# Autodesk Inventor assembly: eh2p-00 - K3D EH2P
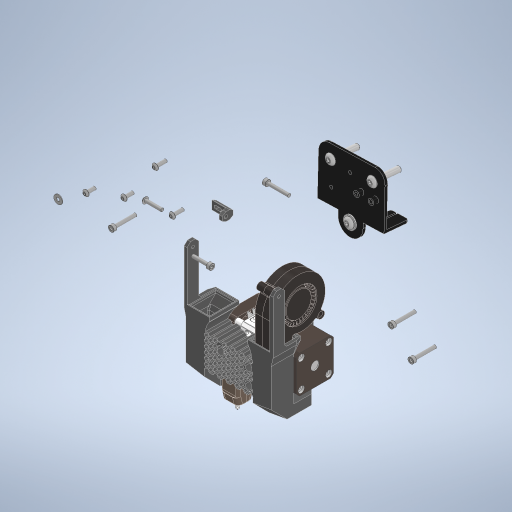
[picture p0: Inventor's stored thumbnail of the model, 512x512]
Saved by Autodesk Inventor 2024 (Build 280153000, 153)
## iProperties
Created: 2023-11-25
Part Number: eh2p-00 - K3D EH2P
Description: CAx-IF Rec.Pracs.---Representation and Presentation of Product Manufacturing Information (PMI)---4.0---2014-10-13
Document SubType Name: Assembly
Designer: wtsh
Sending System: SIEMENS PLM Software NX2306.1700
Preprocessor: ST-DEVELOPER v19.4
Title: eh2p-00 - K3D EH2P
## Documents named in this file (20)
- C:\Users\wtsh\Documents\Inventor\K3D-EHP\k3d_ehp_v2_assembly\k3d_ehp_v2_assembly.iam
- C:\Users\wtsh\Documents\Inventor\K3D-EHP\k3d_ehp_v2_assembly\Screw round M3x6.ipt
- C:\Users\wtsh\Documents\Inventor\K3D-EHP\k3d_ehp_v2_assembly\Screw socket M3x20.ipt
- C:\Users\wtsh\Documents\Inventor\K3D-EHP\k3d_ehp_v2_assembly\Screw round M5x25.ipt
- C:\Users\wtsh\Documents\Inventor\K3D-EHP\k3d_ehp_v2_assembly\eh2p-06b - United fan ducts for v6 with CRTouch.ipt
- C:\Users\wtsh\Documents\Inventor\K3D-EHP\k3d_ehp_v2_assembly\eh2p-06a - United fan ducts for v6.ipt
- C:\Users\wtsh\Documents\Inventor\K3D-EHP\k3d_ehp_v2_assembly\eh2p-05a - United fan ducts for volcano.ipt
- C:\Users\wtsh\Documents\Inventor\K3D-EHP\k3d_ehp_v2_assembly\eh2p-05b - United fan ducts for volcano with CRTouch.ipt
- C:\Users\wtsh\Documents\Inventor\K3D-EHP\k3d_ehp_v2_assembly\CR-Touch.ipt
- C:\Users\wtsh\Documents\Inventor\K3D-EHP\k3d_ehp_v2_assembly\Fan 5015.ipt
- C:\Users\wtsh\Documents\Inventor\K3D-EHP\k3d_ehp_v2_assembly\Screw round M3x16.ipt
- C:\Users\wtsh\Documents\Inventor\K3D-EHP\k3d_ehp_v2_assembly\Screw round M3x8.ipt
- C:\Users\wtsh\Documents\Inventor\K3D-EHP\k3d_ehp_v2_assembly\Nut M3.ipt
- C:\Users\wtsh\Documents\Inventor\K3D-EHP\k3d_ehp_v2_assembly\Washer M3.ipt
- C:\Users\wtsh\Documents\Inventor\K3D-EHP\k3d_ehp_v2_assembly\eh2p-02 - mount slider.ipt
- C:\Users\wtsh\Documents\Inventor\K3D-EHP\k3d_ehp_v2_assembly\h2 v2s lite.ipt
- C:\Users\wtsh\Documents\Inventor\K3D-EHP\k3d_ehp_v2_assembly\Washer M5.ipt
- C:\Users\wtsh\Documents\Inventor\K3D-EHP\k3d_ehp_v2_assembly\Screw round M3x10.ipt
- C:\Users\wtsh\Documents\Inventor\K3D-EHP\k3d_ehp_v2_assembly\eh2p-01 - H2 V2S mount (ender).ipt
- C:\Users\wtsh\Documents\Inventor\K3D-EHP\k3d_ehp_v2_assembly\Ender-3 carriage.ipt
## Components (30 placed, 19 different names)
1. Screw round M3x6 — С поворотом:1
2. Screw round M3x6:1 — С поворотом:6
3. Screw socket M3x20
4. Screw socket M3x20:1
5. Screw round M5x25 — С поворотом:5
6. Screw round M5x25:1 — С поворотом:2
7. eh2p-06b - United fan ducts for v6 with CRTouch — Жесткий:1, Совмещение:1, Угол:3, Совмещение:2, С поворотом:8
8. eh2p-06a - United fan ducts for v6
9. eh2p-05a - United fan ducts for volcano
10. eh2p-05b - United fan ducts for volcano with CRTouch
11. CR-Touch — Жесткий:1
12. Fan 5015 — С поворотом:8
13. Fan 5015:1
14. Screw socket M3x20:2
15. Screw socket M3x20:3
16. Screw socket M3x20:4
17. Screw round M3x16
18. Screw round M3x8
19. Nut M3
20. Washer M3
21. eh2p-02 - mount slider
22. h2 v2s lite — С поворотом:7, Угол:2, Совмещение:1, Угол:3, Совмещение:2
23. Screw round M5x25:2 — С поворотом:3
24. Washer M5 — С поворотом:3, С поворотом:4
25. Screw round M3x10
26. Screw round M3x10:1
27. Screw round M3x8:1
28. Screw round M3x8:2
29. eh2p-01 - H2 V2S mount (ender) — С поворотом:1, Угол:1, С поворотом:6, С поворотом:7, Угол:2
30. Ender-3 carriage — С поворотом:2, С поворотом:4, С поворотом:5
## Relationships (14: RevoluteJoint 8, Angle 3, Mate 2, WeldJoint 1)
- Жесткий:1 [WeldJoint]: eh2p-06b - United fan ducts for v6 with CRTouch ↔ CR-Touch
- С поворотом:1 [RevoluteJoint]: Screw round M3x6 ↔ eh2p-01 - H2 V2S mount (ender)
- Угол:1 [Angle] (180 deg): eh2p-01 - H2 V2S mount (ender)
- С поворотом:2 [RevoluteJoint]: Screw round M5x25:1 ↔ Ender-3 carriage
- С поворотом:3 [RevoluteJoint]: Screw round M5x25:2 ↔ Washer M5
- С поворотом:4 [RevoluteJoint]: Washer M5 ↔ Ender-3 carriage
- С поворотом:5 [RevoluteJoint]: Screw round M5x25 ↔ Ender-3 carriage
- С поворотом:6 [RevoluteJoint]: Screw round M3x6:1 ↔ eh2p-01 - H2 V2S mount (ender)
- С поворотом:7 [RevoluteJoint]: h2 v2s lite ↔ eh2p-01 - H2 V2S mount (ender)
- Угол:2 [Angle] (180 deg): h2 v2s lite ↔ eh2p-01 - H2 V2S mount (ender)
- Совмещение:1 [Mate]: eh2p-06b - United fan ducts for v6 with CRTouch ↔ h2 v2s lite
- Угол:3 [Angle] (0 deg): eh2p-06b - United fan ducts for v6 with CRTouch ↔ h2 v2s lite
- Совмещение:2 [Mate]: eh2p-06b - United fan ducts for v6 with CRTouch ↔ h2 v2s lite
- С поворотом:8 [RevoluteJoint]: eh2p-06b - United fan ducts for v6 with CRTouch ↔ Fan 5015
